# Autodesk Inventor assembly: elevator
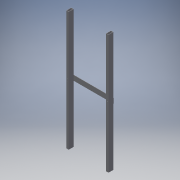
[picture p0: Inventor's stored thumbnail of the model, 180x180]
Saved by Autodesk Inventor 2017 (Build 210142000, 142)
## iProperties
Created: 2017-12-27
Part Number: elevator
Document SubType Name: Assembly
Designer: Micah
Author: Micah
## Documents named in this file (3)
- C:\Users\Micah\Desktop\inventor\CADathon-2017\Assemblies\elevator.iam
- C:\Users\Micah\Desktop\inventor\CADathon-2017\Parts\Elevator\crossbeam.ipt
- C:\Users\Micah\Desktop\inventor\CADathon-2017\Parts\Elevator\main beam.ipt
## Components (3 placed, 2 different names)
1. crossbeam:1 — Mate:1, Mate:2
2. main beam:1 — Mate:1
3. main beam:2 — Mate:2
## Relationships (2: Mate 2)
- Mate:1: crossbeam:1 ↔ main beam:1
- Mate:2: crossbeam:1 ↔ main beam:2
